# Autodesk Inventor assembly: HAND_asm2
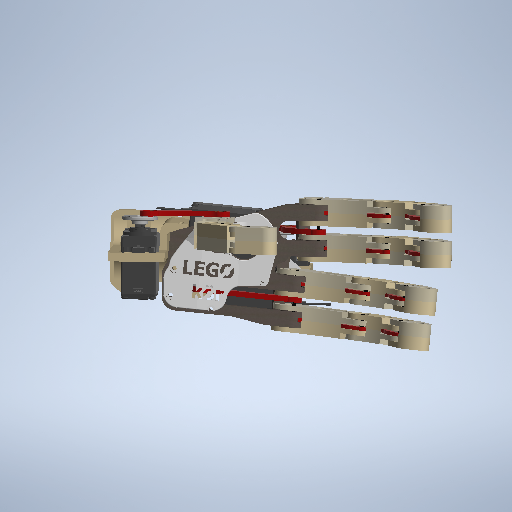
[picture p0: Inventor's stored thumbnail of the model, 512x512]
Saved by Autodesk Inventor 2025.2 (Build 292293000, 293)
## iProperties
Part Number: HAND_asm2
Document SubType Name: Assembly
Designer: esandor
Author: esandor
## Documents named in this file (23)
- C:\Users\esandor\Documents\Inventor\Workspace\LEGO_GITHUB_INDACT_CAD\HAND_main_modell.iam
- C:\Users\esandor\Documents\Inventor\Workspace\LEGO_GITHUB_INDACT_CAD\PALM\PALM_B.ipt
- C:\Users\esandor\Documents\Inventor\Workspace\LEGO_GITHUB_INDACT_CAD\HAND\HAND_DDP.ipt
- C:\Users\esandor\Documents\Inventor\Workspace\LEGO_GITHUB_INDACT_CAD\FINGER\FIN_PP_T.ipt
- C:\Users\esandor\Documents\Inventor\Workspace\LEGO_GITHUB_INDACT_CAD\FINGER\FIN_DP_L.ipt
- C:\Users\esandor\Documents\Inventor\Workspace\LEGO_GITHUB_INDACT_CAD\FINGER\FIN_PP_B.ipt
- C:\Users\esandor\Documents\Inventor\Workspace\LEGO_GITHUB_INDACT_CAD\FINGER\FIN_PM_T.ipt
- C:\Users\esandor\Documents\Inventor\Workspace\LEGO_GITHUB_INDACT_CAD\FINGER\FIN_PM_B.ipt
- C:\Users\esandor\Documents\Inventor\Workspace\LEGO_GITHUB_INDACT_CAD\FINGER\FIN_DP_S.ipt
- C:\Users\esandor\Documents\Inventor\Workspace\LEGO_GITHUB_INDACT_CAD\FINGER\FIN_PD_T.ipt
- C:\Users\esandor\Documents\Inventor\Workspace\LEGO_GITHUB_INDACT_CAD\FINGER\FIN_PD_B.ipt
- C:\Users\esandor\Documents\Inventor\Workspace\LEGO_GITHUB_INDACT_CAD\FINGER\FIN_MP.ipt
- C:\Users\esandor\Documents\Inventor\Workspace\LEGO_GITHUB_INDACT_CAD\FINGER\FIN_MD.ipt
- C:\Users\esandor\Documents\Inventor\Workspace\LEGO_GITHUB_INDACT_CAD\PALM\PALM_L.ipt
- C:\Users\esandor\Documents\Inventor\Workspace\LEGO_GITHUB_INDACT_CAD\PALM\PALM_MH_L.ipt
- C:\Users\esandor\Documents\Inventor\Workspace\LEGO_GITHUB_INDACT_CAD\PALM\PALM_MH_U.ipt
- C:\Users\esandor\Documents\Inventor\Workspace\LEGO_GITHUB_INDACT_CAD\HAND\HAND_MO.ipt
- C:\Users\esandor\Documents\Inventor\Workspace\LEGO_GITHUB_INDACT_CAD\HAND\HAND_MOG.ipt
- C:\Users\esandor\Documents\Inventor\Workspace\LEGO_GITHUB_INDACT_CAD\HAND\HAND_PH.ipt
- C:\Users\esandor\Documents\Inventor\Workspace\LEGO_GITHUB_INDACT_CAD\HAND\HAND_FL.ipt
- C:\Users\esandor\Documents\Inventor\Workspace\LEGO_GITHUB_INDACT_CAD\HAND\HAND_M_LF.ipt
- C:\Users\esandor\Documents\Inventor\Workspace\LEGO_GITHUB_INDACT_CAD\HAND\HAND_M_TF.ipt
- C:\Users\esandor\Documents\Inventor\Workspace\LEGO_GITHUB_INDACT_CAD\HAND\HAND_M_IF.ipt
## Components (81 placed, 22 different names)
1. PALM_B:1 — Mate:2, Tangent:2, Insert:2, Insert:9, Insert:11, Mate:24, Tangent:44, Mate:25, Insert:30, Insert:31, Mate:28, Insert:32, Insert:33, Tangent:63, Mate:36, Insert:42, Insert:43, Mate:37, Insert:44, Insert:45
2. FIN_DP_S:1 — Insert:2, Tangent:5
3. FIN_PP_T:1 — Mate:1, Insert:1, Tangent:1, Mate:2, Tangent:2, Insert:4, Mate:4, Insert:5, Mate:5
4. FIN_PP_B:1 — Mate:1, Insert:1, Tangent:1, Tangent:21
5. FIN_DP_S:2 — Insert:4, Tangent:9
6. FIN_PM_T:1 — Mate:3, Tangent:3, Tangent:4, Mate:4, Insert:5, Insert:6, Insert:7, Mate:7
7. FIN_PM_B:1 — Mate:3, Tangent:3, Tangent:4, Angle:1
8. FIN_DP_L:2 — Insert:6, Tangent:6
9. FIN_MP:1 — Tangent:5, Mate:5, Tangent:6
10. FIN_PD_T:1 — Mate:6, Tangent:7, Tangent:8, Insert:7, Insert:8
11. FIN_PD_B:1 — Mate:6, Tangent:7, Tangent:8, Angle:2
12. FIN_DP_L:3 — Insert:8, Tangent:10
13. FIN_MD:1 — Mate:7, Tangent:9, Tangent:10
14. FIN_PP_T:2 — Tangent:11, Tangent:12, Mate:8, Insert:9, Insert:12, Insert:13, Mate:10, Insert:17
15. FIN_PP_B:2 — Tangent:11, Tangent:12, Mate:8, Mate:49
16. FIN_DP_S:3 — Insert:11, Tangent:15
17. FIN_DP_S:4 — Insert:12, Tangent:19
18. FIN_PM_T:2 — Insert:13, Insert:14, Insert:15, Mate:12
19. FIN_PM_B:2 — Angle:1
20. FIN_DP_L:5 — Insert:14, Tangent:16
21. FIN_MP:2 — Mate:10, Tangent:15, Tangent:16
22. FIN_PD_T:2 — Insert:15, Insert:16
23. FIN_PD_B:2 — Angle:2
24. FIN_DP_L:6 — Insert:16, Tangent:20
25. FIN_MD:3 — Tangent:19, Mate:12, Tangent:20
26. HAND_DDP:3 — Insert:17, Tangent:21, Tangent:65
27. FIN_PP_T:3 — Mate:25, Mate:26, Mate:52
28. FIN_PP_B:3 — Tangent:63
29. FIN_DP_S:6
30. FIN_PM_T:3
31. FIN_PM_B:3
32. FIN_DP_L:7 — Tangent:48
33. FIN_PD_T:3
34. FIN_PD_B:3
35. FIN_DP_L:8
36. FIN_MD:4
37. FIN_PP_T:4 — Mate:24, Tangent:44, Mate:27
38. FIN_PP_B:4
39. FIN_DP_S:8
40. FIN_PM_T:4
41. FIN_PM_B:4
42. FIN_DP_L:9 — Tangent:50
43. FIN_PD_T:4
44. FIN_PD_B:4
45. FIN_DP_L:10
46. FIN_MD:5
47. HAND_DDP:4 — Tangent:67
48. FIN_DP_S:9 — Insert:30, Tangent:47
49. FIN_MP:3 — Mate:26, Tangent:47, Tangent:48
50. FIN_DP_S:10 — Insert:31, Tangent:49
51. FIN_MP:4 — Mate:27, Tangent:49, Tangent:50
52. PALM_L:1 — Mate:28, Insert:32, Insert:33, Mate:35, Insert:40, Insert:41
53. FIN_PP_T:5 — Insert:54
54. FIN_PP_B:5 — Mate:35, Insert:40
55. FIN_DP_S:12
56. FIN_PM_T:5
57. FIN_PM_B:5
58. FIN_DP_L:11
59. FIN_MP:5 — Tangent:62
60. FIN_PD_T:5
61. FIN_PD_B:5
62. FIN_DP_L:12
63. FIN_MD:6
64. FIN_DP_S:13 — Insert:41, Tangent:62
65. PALM_MH_L:1 — Mate:36, Insert:42, Insert:43, Mate:40, Insert:55, Insert:56
66. PALM_MH_U:1 — Mate:37, Insert:44, Insert:45, Mate:38, Insert:46, Insert:47, Mate:39, Insert:48, Insert:49
67. HAND_MO:1 — Mate:38, Insert:46, Insert:47, Rotational:2
68. HAND_MO:2 — Mate:39, Insert:48, Insert:49, Rotational:1
69. HAND_MO:3 — Mate:40, Insert:55, Insert:56, Rotational:3
70. HAND_MOG:1 — Rotational:1, Tangent:70
71. HAND_PH:1 — Tangent:64, Flush:1, Tangent:65
72. HAND_FL:1 — Mate:50, Mate:51, Tangent:68
73. HAND_M_LF:1 — Mate:50, Mate:51, Tangent:66, Flush:2, Mate:52
74. HAND_M_TF:1 — Mate:44, Mate:45, Mate:46, Tangent:71
75. HAND_FL:2 — Mate:44, Tangent:70, Tangent:71
76. HAND_FL:3 — Mate:45, Mate:46, Insert:54
77. HAND_M_IF:1 — Mate:47, Mate:48, Tangent:64, Flush:1, Mate:49
78. HAND_FL:4 — Mate:47, Mate:48, Tangent:69
79. HAND_PH:2 — Tangent:66, Flush:2, Tangent:67
80. HAND_MOG:2 — Rotational:2, Tangent:69
81. HAND_MOG:3 — Rotational:3, Tangent:68
## Relationships (164: Tangent 60, Insert 50, Mate 47, RevoluteJoint 3, Angle 2, Flush 2)
- Mate:1: FIN_PP_T:1 ↔ FIN_PP_B:1
- Insert:1: FIN_PP_T:1 ↔ FIN_PP_B:1
- Tangent:1: FIN_PP_T:1 ↔ FIN_PP_B:1
- Mate:2: PALM_B:1 ↔ FIN_PP_T:1
- Tangent:2: PALM_B:1 ↔ FIN_PP_T:1
- Insert:2: PALM_B:1 ↔ FIN_DP_S:1
- Insert:4: FIN_PP_T:1 ↔ FIN_DP_S:2
- Mate:3: FIN_PM_T:1 ↔ FIN_PM_B:1
- Tangent:3: FIN_PM_T:1 ↔ FIN_PM_B:1
- Tangent:4: FIN_PM_T:1 ↔ FIN_PM_B:1
- Mate:4: FIN_PP_T:1 ↔ FIN_PM_T:1
- Insert:5: FIN_PP_T:1 ↔ FIN_PM_T:1
- Insert:6: FIN_PM_T:1 ↔ FIN_DP_L:2
- Tangent:5: FIN_DP_S:1 ↔ FIN_MP:1
- Mate:5: FIN_PP_T:1 ↔ FIN_MP:1
- Tangent:6: FIN_DP_L:2 ↔ FIN_MP:1
- Mate:6: FIN_PD_T:1 ↔ FIN_PD_B:1
- Tangent:7: FIN_PD_T:1 ↔ FIN_PD_B:1
- Tangent:8: FIN_PD_T:1 ↔ FIN_PD_B:1
- Insert:7: FIN_PM_T:1 ↔ FIN_PD_T:1
- Insert:8: FIN_PD_T:1 ↔ FIN_DP_L:3
- Mate:7: FIN_PM_T:1 ↔ FIN_MD:1
- Tangent:9: FIN_DP_S:2 ↔ FIN_MD:1
- Tangent:10: FIN_DP_L:3 ↔ FIN_MD:1
- Tangent:11: FIN_PP_T:2 ↔ FIN_PP_B:2
- Tangent:12: FIN_PP_T:2 ↔ FIN_PP_B:2
- Mate:8: FIN_PP_T:2 ↔ FIN_PP_B:2
- Insert:9: PALM_B:1 ↔ FIN_PP_T:2
- Insert:11: PALM_B:1 ↔ FIN_DP_S:3
- Insert:12: FIN_PP_T:2 ↔ FIN_DP_S:4
- [Mate]: FIN_PM_T:2 ↔ FIN_PM_B:2
- [Tangent]: FIN_PM_T:2 ↔ FIN_PM_B:2
- [Tangent]: FIN_PM_T:2 ↔ FIN_PM_B:2
- Insert:13: FIN_PP_T:2 ↔ FIN_PM_T:2
- Insert:14: FIN_PM_T:2 ↔ FIN_DP_L:5
- Mate:10: FIN_PP_T:2 ↔ FIN_MP:2
- Tangent:15: FIN_DP_S:3 ↔ FIN_MP:2
- Tangent:16: FIN_DP_L:5 ↔ FIN_MP:2
- [Mate]: FIN_PD_T:2 ↔ FIN_PD_B:2
- [Tangent]: FIN_PD_T:2 ↔ FIN_PD_B:2
- [Tangent]: FIN_PD_T:2 ↔ FIN_PD_B:2
- Insert:15: FIN_PM_T:2 ↔ FIN_PD_T:2
- Insert:16: FIN_PD_T:2 ↔ FIN_DP_L:6
- Tangent:19: FIN_DP_S:4 ↔ FIN_MD:3
- Mate:12: FIN_PM_T:2 ↔ FIN_MD:3
- Tangent:20: FIN_DP_L:6 ↔ FIN_MD:3
- Insert:17 (-0.43 mm): FIN_PP_T:2 ↔ HAND_DDP:3
- Tangent:21: FIN_PP_B:1 ↔ HAND_DDP:3
- [Mate]: FIN_PP_T:3 ↔ FIN_PP_B:3
- [Insert]: FIN_PP_T:3 ↔ FIN_PP_B:3
- [Tangent]: FIN_PP_T:3 ↔ FIN_PP_B:3
- [Insert]: FIN_PP_T:3 ↔ FIN_DP_S:6
- [Mate]: FIN_PM_T:3 ↔ FIN_PM_B:3
- [Tangent]: FIN_PM_T:3 ↔ FIN_PM_B:3
- [Tangent]: FIN_PM_T:3 ↔ FIN_PM_B:3
- [Mate]: FIN_PP_T:3 ↔ FIN_PM_T:3
- [Insert]: FIN_PP_T:3 ↔ FIN_PM_T:3
- [Insert]: FIN_PM_T:3 ↔ FIN_DP_L:7
- [Mate]: FIN_PD_T:3 ↔ FIN_PD_B:3
- [Tangent]: FIN_PD_T:3 ↔ FIN_PD_B:3
- [Tangent]: FIN_PD_T:3 ↔ FIN_PD_B:3
- [Insert]: FIN_PM_T:3 ↔ FIN_PD_T:3
- [Insert]: FIN_PD_T:3 ↔ FIN_DP_L:8
- [Mate]: FIN_PM_T:3 ↔ FIN_MD:4
- [Tangent]: FIN_DP_S:6 ↔ FIN_MD:4
- [Tangent]: FIN_DP_L:8 ↔ FIN_MD:4
- [Tangent]: FIN_PP_T:4 ↔ FIN_PP_B:4
- [Tangent]: FIN_PP_T:4 ↔ FIN_PP_B:4
- [Mate]: FIN_PP_T:4 ↔ FIN_PP_B:4
- [Insert]: FIN_PP_T:4 ↔ FIN_DP_S:8
- [Mate]: FIN_PM_T:4 ↔ FIN_PM_B:4
- [Tangent]: FIN_PM_T:4 ↔ FIN_PM_B:4
- [Tangent]: FIN_PM_T:4 ↔ FIN_PM_B:4
- [Insert]: FIN_PP_T:4 ↔ FIN_PM_T:4
- [Insert]: FIN_PM_T:4 ↔ FIN_DP_L:9
- [Mate]: FIN_PD_T:4 ↔ FIN_PD_B:4
- [Tangent]: FIN_PD_T:4 ↔ FIN_PD_B:4
- [Tangent]: FIN_PD_T:4 ↔ FIN_PD_B:4
- [Insert]: FIN_PM_T:4 ↔ FIN_PD_T:4
- [Insert]: FIN_PD_T:4 ↔ FIN_DP_L:10
- [Tangent]: FIN_DP_S:8 ↔ FIN_MD:5
- [Mate]: FIN_PM_T:4 ↔ FIN_MD:5
- [Tangent]: FIN_DP_L:10 ↔ FIN_MD:5
- [Insert] (-0.43 mm): FIN_PP_T:4 ↔ HAND_DDP:4
- [Tangent]: FIN_PP_B:3 ↔ HAND_DDP:4
- Mate:24: PALM_B:1 ↔ FIN_PP_T:4
- Tangent:44: PALM_B:1 ↔ FIN_PP_T:4
- Mate:25: PALM_B:1 ↔ FIN_PP_T:3
- Insert:30: PALM_B:1 ↔ FIN_DP_S:9
- Mate:26: FIN_PP_T:3 ↔ FIN_MP:3
- Tangent:47: FIN_DP_S:9 ↔ FIN_MP:3
- Tangent:48: FIN_DP_L:7 ↔ FIN_MP:3
- Insert:31: PALM_B:1 ↔ FIN_DP_S:10
- Mate:27: FIN_PP_T:4 ↔ FIN_MP:4
- Tangent:49: FIN_DP_S:10 ↔ FIN_MP:4
- Tangent:50: FIN_DP_L:9 ↔ FIN_MP:4
- Mate:28: PALM_B:1 ↔ PALM_L:1
- Insert:32: PALM_B:1 ↔ PALM_L:1
- Insert:33: PALM_B:1 ↔ PALM_L:1
- [Mate]: FIN_PP_T:5 ↔ FIN_PP_B:5
- [Insert]: FIN_PP_T:5 ↔ FIN_PP_B:5
- [Tangent]: FIN_PP_T:5 ↔ FIN_PP_B:5
- [Insert]: FIN_PP_T:5 ↔ FIN_DP_S:12
- [Mate]: FIN_PM_T:5 ↔ FIN_PM_B:5
- [Tangent]: FIN_PM_T:5 ↔ FIN_PM_B:5
- [Tangent]: FIN_PM_T:5 ↔ FIN_PM_B:5
- [Mate]: FIN_PP_T:5 ↔ FIN_PM_T:5
- [Insert]: FIN_PP_T:5 ↔ FIN_PM_T:5
- [Insert]: FIN_PM_T:5 ↔ FIN_DP_L:11
- [Mate]: FIN_PP_T:5 ↔ FIN_MP:5
- [Tangent]: FIN_DP_L:11 ↔ FIN_MP:5
- [Mate]: FIN_PD_T:5 ↔ FIN_PD_B:5
- [Tangent]: FIN_PD_T:5 ↔ FIN_PD_B:5
- [Tangent]: FIN_PD_T:5 ↔ FIN_PD_B:5
- [Insert]: FIN_PM_T:5 ↔ FIN_PD_T:5
- [Insert]: FIN_PD_T:5 ↔ FIN_DP_L:12
- [Mate]: FIN_PM_T:5 ↔ FIN_MD:6
- [Tangent]: FIN_DP_S:12 ↔ FIN_MD:6
- [Tangent]: FIN_DP_L:12 ↔ FIN_MD:6
- Mate:35: PALM_L:1 ↔ FIN_PP_B:5
- Insert:40: PALM_L:1 ↔ FIN_PP_B:5
- Insert:41: PALM_L:1 ↔ FIN_DP_S:13
- Tangent:62: FIN_MP:5 ↔ FIN_DP_S:13
- Tangent:63: PALM_B:1 ↔ FIN_PP_B:3
- Angle:1 (0 deg): FIN_PM_B:1 ↔ FIN_PM_B:2
- Angle:2 (0 deg): FIN_PD_B:1 ↔ FIN_PD_B:2
- Mate:36: PALM_B:1 ↔ PALM_MH_L:1
- Insert:42: PALM_B:1 ↔ PALM_MH_L:1
- Insert:43: PALM_B:1 ↔ PALM_MH_L:1
- Mate:37: PALM_B:1 ↔ PALM_MH_U:1
- Insert:44: PALM_B:1 ↔ PALM_MH_U:1
- Insert:45: PALM_B:1 ↔ PALM_MH_U:1
- Mate:38: PALM_MH_U:1 ↔ HAND_MO:1
- Insert:46: PALM_MH_U:1 ↔ HAND_MO:1
- Insert:47: PALM_MH_U:1 ↔ HAND_MO:1
- Mate:39: PALM_MH_U:1 ↔ HAND_MO:2
- Insert:48: PALM_MH_U:1 ↔ HAND_MO:2
- Insert:49: PALM_MH_U:1 ↔ HAND_MO:2
- Mate:40: PALM_MH_L:1 ↔ HAND_MO:3
- Mate:44: HAND_M_TF:1 ↔ HAND_FL:2
- Mate:45: HAND_M_TF:1 ↔ HAND_FL:3
- Mate:46: HAND_M_TF:1 ↔ HAND_FL:3
- Insert:54: FIN_PP_T:5 ↔ HAND_FL:3
- Mate:47: HAND_M_IF:1 ↔ HAND_FL:4
- Mate:48: HAND_M_IF:1 ↔ HAND_FL:4
- Tangent:64: HAND_PH:1 ↔ HAND_M_IF:1
- Flush:1: HAND_PH:1 ↔ HAND_M_IF:1
- Tangent:65: HAND_DDP:3 ↔ HAND_PH:1
- Mate:49: FIN_PP_B:2 ↔ HAND_M_IF:1
- Mate:50: HAND_FL:1 ↔ HAND_M_LF:1
- Mate:51: HAND_FL:1 ↔ HAND_M_LF:1
- Tangent:66: HAND_M_LF:1 ↔ HAND_PH:2
- Flush:2: HAND_M_LF:1 ↔ HAND_PH:2
- Tangent:67: HAND_DDP:4 ↔ HAND_PH:2
- Mate:52: FIN_PP_T:3 ↔ HAND_M_LF:1
- Insert:55: PALM_MH_L:1 ↔ HAND_MO:3
- Insert:56: PALM_MH_L:1 ↔ HAND_MO:3
- Tangent:68: HAND_FL:1 ↔ HAND_MOG:3
- Tangent:69: HAND_FL:4 ↔ HAND_MOG:2
- Tangent:70: HAND_MOG:1 ↔ HAND_FL:2
- Tangent:71: HAND_M_TF:1 ↔ HAND_FL:2
- Rotational:1 [RevoluteJoint]: HAND_MO:2 ↔ HAND_MOG:1
- Rotational:2 [RevoluteJoint]: HAND_MO:1 ↔ HAND_MOG:2
- Rotational:3 [RevoluteJoint]: HAND_MO:3 ↔ HAND_MOG:3
## Named parameters: d143_d117 = 0 mm, d144_d119 = 0 mm, d145_d120 = 0 mm, d151_d127 = 0 mm, d152_d128 = 0 mm, d153_d129 = 0 mm, d263_d161 = 0 mm, d265_d132 = 0 mm, d266_d133 = 0 mm, d267_d134 = 0 mm, d268_d136 = 0 mm, d269_d137 = 0 mm, d270_d138 = 0 mm, d271_d142 = 0 mm, d272_d143_d117 = 0 mm, d273_d144_d119 = 0 mm, d274_d145_d120 = 0 mm, d275_d146 = 0 mm, d276_d147 = 0 mm, d280_d151_d127 = 0 mm, d281_d152_d128 = 0 mm, d282_d153_d129 = 0 mm, d283_d154 = 0 mm, d284_d155 = 0 mm, d285_d156 = 0 mm, d286_d157 = 0 mm, d287_d158 = 0 mm, d288_d160 = -0.43 mm, d289_d108 = 0 mm, d290_d109 = 0 mm, d291_d110 = 0 mm, d292_d116 = 0 mm, d293_d117 = 0 mm, d294_d119 = 0 mm, d295_d120 = 0 mm, d296_d121 = 0 mm, d297_d122 = 0 mm, d298_d123 = 0 mm, d302_d127 = 0 mm, d303_d128 = 0 mm, d304_d129 = 0 mm, d305_d130 = 0 mm, d306_d131 = 0 mm, d325_d132 = 0 mm, d326_d133 = 0 mm, d327_d134 = 0 mm, d328_d108 = 0 mm, d329_d109 = 0 mm, d330_d110 = 0 mm, d331_d116 = 0 mm, d332_d117 = 0 mm, d333_d119 = 0 mm, d334_d120 = 0 mm, d335_d121 = 0 mm, d336_d122 = 0 mm, d337_d123 = 0 mm, d339_d125 = 0 mm, d340_d126 = 0 mm, d341_d127 = 0 mm, d342_d128 = 0 mm, d343_d129 = 0 mm, d344_d130 = 0 mm, d345_d131 = 0 mm
